# Autodesk Inventor assembly: Ramp Assembly
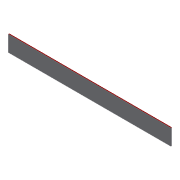
[picture p0: Inventor's stored thumbnail of the model, 180x180]
Saved by Autodesk Inventor 2015 (Build 190159000, 159)
## iProperties
Created: 2015-01-19
Part Number: Ramp Assembly
Document SubType Name: Assembly
Designer: Peter
Author: Peter
## Documents named in this file (3)
- T:\FILES\FIRST-Team-1719-CAD-Team\2015 Playing Field\Team 1719 Practice Field\Scoring Platform - Construction Design\Ramp Assembly.iam
- T:\FILES\FIRST-Team-1719-CAD-Team\2015 Playing Field\Team 1719 Practice Field\Scoring Platform - Construction Design\Plywood Ramp 375.ipt
- T:\FILES\FIRST-Team-1719-CAD-Team\2015 Playing Field\Team 1719 Practice Field\Scoring Platform - Construction Design\Clear Ramp Surface 125.ipt
## Components (2 placed, 2 different names)
1. Plywood Ramp 375:1 — Mate:1, Flush:1, Flush:2
2. Clear Ramp Surface 125:1 — Mate:1, Flush:1, Flush:2
## Relationships (3: Flush 2, Mate 1)
- Mate:1: Plywood Ramp 375:1 ↔ Clear Ramp Surface 125:1
- Flush:1: Plywood Ramp 375:1 ↔ Clear Ramp Surface 125:1
- Flush:2: Plywood Ramp 375:1 ↔ Clear Ramp Surface 125:1
